# Autodesk Inventor assembly: New_large_hinge_assembly
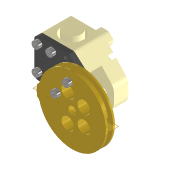
[picture p0: Inventor's stored thumbnail of the model, 180x180]
Saved by Autodesk Inventor 2022 (Build 260153000, 153)
## iProperties
Created: 2022-07-14
Part Number: New_large_hinge_assembly
Document SubType Name: Assembly
Designer: dell
Author: dell
## Documents named in this file (6)
- D:\xxxx\Uni\Part IV\MECHENG_700\Part_IV_project_CAD\Bird_skeleton_prototypes\Wing_drone_V1\Bird_wing_V2\New_large_hinge_assembly.iam
- D:\xxxx\Uni\Part IV\MECHENG_700\Part_IV_project_CAD\Bird_skeleton_prototypes\Wing_drone_V1\Bird_wing_V2\New_hinge.ipt
- D:\xxxx\Uni\Part IV\MECHENG_700\Part_IV_project_CAD\Bird_skeleton_prototypes\Wing_drone_V1\Bird_wing_V2\New_hinge_plate.ipt
- D:\xxxx\Uni\Part IV\MECHENG_700\Part_IV_project_CAD\Bird_skeleton_prototypes\Wing_drone_V1\Bird_wing_V2\New_coupling_pulley_p1.ipt
- D:\xxxx\Uni\Part IV\MECHENG_700\Part_IV_project_CAD\Bird_skeleton_prototypes\Wing_drone_V1\Bird_wing_V2\New_coupling_pulley_p2.ipt
- D:\xxxx\Uni\Part IV\MECHENG_700\Part_IV_project_CAD\Bird_skeleton_prototypes\Wing_drone_V1\Bird_wing_V2\M2_bolt.ipt
## Components (11 placed, 5 different names)
1. New_hinge:1 — Mate:1, Mate:2, Mate:6, Mate:7, Mate:8
2. New_hinge:2 — Mate:1, Mate:2, Mate:3, Mate:4, Mate:5
3. New_hinge_plate:3 — Mate:3, Mate:4, Mate:5, Mate:12, Mate:13, Mate:14
4. New_hinge_plate:4 — Mate:6, Mate:7, Mate:8, Mate:15, Mate:16, Mate:17, Mate:22, Mate:23, Mate:24, Mate:25, Mate:26, Mate:27
5. New_coupling_pulley_p1:2 — Mate:12, Mate:13, Mate:14
6. New_coupling_pulley_p2:1 — Mate:15, Mate:16, Mate:17, Mate:18, Mate:19, Mate:20, Mate:21
7. M2_bolt:1 — Mate:18, Mate:20
8. M2_bolt:2 — Mate:19, Mate:21
9. M2_bolt:3 — Mate:24, Mate:27
10. M2_bolt:4 — Mate:23, Mate:26
11. M2_bolt:5 — Mate:22, Mate:25
## Relationships (24: Mate 24)
- Mate:1: New_hinge:1 ↔ New_hinge:2
- Mate:2: New_hinge:1 ↔ New_hinge:2
- Mate:3: New_hinge:2 ↔ New_hinge_plate:3
- Mate:4: New_hinge:2 ↔ New_hinge_plate:3
- Mate:5: New_hinge:2 ↔ New_hinge_plate:3
- Mate:6: New_hinge:1 ↔ New_hinge_plate:4
- Mate:7: New_hinge:1 ↔ New_hinge_plate:4
- Mate:8: New_hinge:1 ↔ New_hinge_plate:4
- Mate:12: New_hinge_plate:3 ↔ New_coupling_pulley_p1:2
- Mate:13: New_hinge_plate:3 ↔ New_coupling_pulley_p1:2
- Mate:14: New_hinge_plate:3 ↔ New_coupling_pulley_p1:2
- Mate:15: New_hinge_plate:4 ↔ New_coupling_pulley_p2:1
- Mate:16: New_hinge_plate:4 ↔ New_coupling_pulley_p2:1
- Mate:17: New_hinge_plate:4 ↔ New_coupling_pulley_p2:1
- Mate:18: New_coupling_pulley_p2:1 ↔ M2_bolt:1
- Mate:19: New_coupling_pulley_p2:1 ↔ M2_bolt:2
- Mate:20: New_coupling_pulley_p2:1 ↔ M2_bolt:1
- Mate:21: New_coupling_pulley_p2:1 ↔ M2_bolt:2
- Mate:22: New_hinge_plate:4 ↔ M2_bolt:5
- Mate:23: New_hinge_plate:4 ↔ M2_bolt:4
- Mate:24: New_hinge_plate:4 ↔ M2_bolt:3
- Mate:25: New_hinge_plate:4 ↔ M2_bolt:5
- Mate:26: New_hinge_plate:4 ↔ M2_bolt:4
- Mate:27: New_hinge_plate:4 ↔ M2_bolt:3
